# Autodesk Inventor assembly: Tred Link
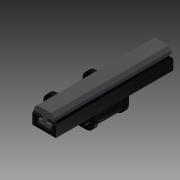
[picture p0: Inventor's stored thumbnail of the model, 180x180]
Saved by Autodesk Inventor 2015 (Build 190159000, 159)
## iProperties
Created: 2012-12-07
Part Number: Tred Link
Document SubType Name: Assembly
Designer: zagerst
Author: zagerst
## Documents named in this file (5)
- C:\Users\nojessen\Documents\GitHub\CAD\COTSParts\Tetrix\Tank Treads\Tred Link.iam
- C:\Users\nojessen\Documents\GitHub\CAD\COTSParts\Tetrix\Tank Treads\TETRIX_TT_LINK_1_2011.ipt
- C:\Users\nojessen\Documents\GitHub\CAD\COTSParts\Tetrix\Tank Treads\TETRIX_TT_LINK_2_2011.ipt
- C:\Users\nojessen\Documents\GitHub\CAD\COTSParts\Tetrix\Tank Treads\TETRIX_TT_LINK_4_2011.ipt
- C:\Users\nojessen\Documents\GitHub\CAD\COTSParts\Tetrix\Tank Treads\tetrix_tt_rubber_2011.ipt
## Components (4 placed, 4 different names)
1. TETRIX_TT_LINK_1_2011:1 — Insert:4, Mate:5
2. TETRIX_TT_LINK_2_2011:1 — Insert:3, Mate:4
3. TETRIX_TT_LINK_4_2011:1 — Flush:2, Mate:2, Mate:3, Insert:3, Mate:4, Insert:4, Mate:5
4. tetrix_tt_rubber_2011:1 — Flush:2, Mate:2, Mate:3
## Relationships (7: Mate 4, Insert 2, Flush 1)
- Flush:2: TETRIX_TT_LINK_4_2011:1 ↔ tetrix_tt_rubber_2011:1
- Mate:2: TETRIX_TT_LINK_4_2011:1 ↔ tetrix_tt_rubber_2011:1
- Mate:3: TETRIX_TT_LINK_4_2011:1 ↔ tetrix_tt_rubber_2011:1
- Insert:3 (-1.3462 mm): TETRIX_TT_LINK_2_2011:1 ↔ TETRIX_TT_LINK_4_2011:1
- Mate:4: TETRIX_TT_LINK_2_2011:1 ↔ TETRIX_TT_LINK_4_2011:1
- Insert:4 (-1.3462 mm): TETRIX_TT_LINK_1_2011:1 ↔ TETRIX_TT_LINK_4_2011:1
- Mate:5: TETRIX_TT_LINK_1_2011:1 ↔ TETRIX_TT_LINK_4_2011:1
